# Autodesk Inventor assembly: BBM
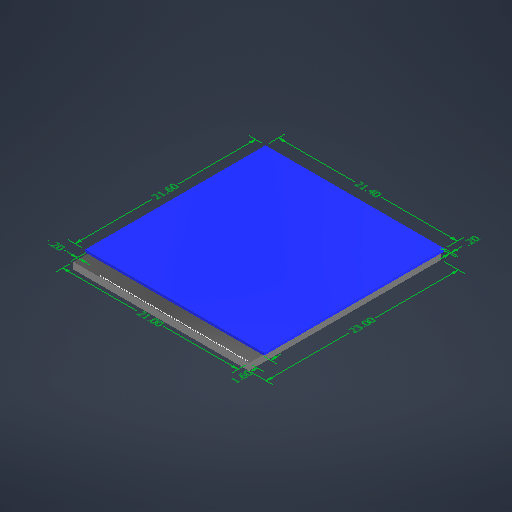
[picture p0: Inventor's stored thumbnail of the model, 512x512]
Saved by Autodesk Inventor 2027 (Build 310192060, 192F)
## iProperties
Created: 2022-02-01
Part Number: BBM
Document SubType Name: Assembly
Designer: Caleb
Author: Caleb
## Documents named in this file (4)
- C:\Users\cfang\Desktop\nebraska-silicon-lab\Hardware\ETL\modules\Tamale v1.7\BBM.iam
- C:\Users\cfang\Desktop\nebraska-silicon-lab\Hardware\ETL\modules\Tamale v1.7\ETL Sensor.ipt
- C:\Users\cfang\Desktop\nebraska-silicon-lab\Hardware\ETL\modules\Tamale v1.7\bump bond.ipt
- C:\Users\cfang\Desktop\nebraska-silicon-lab\Hardware\ETL\modules\Tamale v1.7\ETROC2.ipt
## Components (258 placed, 3 different names)
1. ETL Sensor:1 — Tangent:1, Tangent:2, Tangent:3, Flush:1, Flush:2, Mate:1
2. ETROC2:1 — Flush:1, Flush:2, Mate:1
3. bump bond:1 — Tangent:1, Tangent:2, Tangent:3
4. bump bond:2
5. bump bond:3
6. bump bond:4
7. bump bond:5
8. bump bond:6
9. bump bond:7
10. bump bond:8
11. bump bond:9
12. bump bond:10
13. bump bond:11
14. bump bond:12
15. bump bond:13
16. bump bond:14
17. bump bond:15
18. bump bond:16
19. bump bond:17
20. bump bond:18
21. bump bond:19
22. bump bond:20
23. bump bond:21
24. bump bond:22
25. bump bond:23
26. bump bond:24
27. bump bond:25
28. bump bond:26
29. bump bond:27
30. bump bond:28
31. bump bond:29
32. bump bond:30
33. bump bond:31
34. bump bond:32
35. bump bond:33
36. bump bond:34
37. bump bond:35
38. bump bond:36
39. bump bond:37
40. bump bond:38
41. bump bond:39
42. bump bond:40
43. bump bond:41
44. bump bond:42
45. bump bond:43
46. bump bond:44
47. bump bond:45
48. bump bond:46
49. bump bond:47
50. bump bond:48
51. bump bond:49
52. bump bond:50
53. bump bond:51
54. bump bond:52
55. bump bond:53
56. bump bond:54
57. bump bond:55
58. bump bond:56
59. bump bond:57
60. bump bond:58
61. bump bond:59
62. bump bond:60
63. bump bond:61
64. bump bond:62
65. bump bond:63
66. bump bond:64
67. bump bond:65
68. bump bond:66
69. bump bond:67
70. bump bond:68
71. bump bond:69
72. bump bond:70
73. bump bond:71
74. bump bond:72
75. bump bond:73
76. bump bond:74
77. bump bond:75
78. bump bond:76
79. bump bond:77
80. bump bond:78
81. bump bond:79
82. bump bond:80
83. bump bond:81
84. bump bond:82
85. bump bond:83
86. bump bond:84
87. bump bond:85
88. bump bond:86
89. bump bond:87
90. bump bond:88
91. bump bond:89
92. bump bond:90
93. bump bond:91
94. bump bond:92
95. bump bond:93
96. bump bond:94
97. bump bond:95
98. bump bond:96
99. bump bond:97
100. bump bond:98
101. bump bond:99
102. bump bond:100
103. bump bond:101
104. bump bond:102
105. bump bond:103
106. bump bond:104
107. bump bond:105
108. bump bond:106
109. bump bond:107
110. bump bond:108
111. bump bond:109
112. bump bond:110
113. bump bond:111
114. bump bond:112
115. bump bond:113
116. bump bond:114
117. bump bond:115
118. bump bond:116
119. bump bond:117
120. bump bond:118
121. bump bond:119
122. bump bond:120
123. bump bond:121
124. bump bond:122
125. bump bond:123
126. bump bond:124
127. bump bond:125
128. bump bond:126
129. bump bond:127
130. bump bond:128
131. bump bond:129
132. bump bond:130
133. bump bond:131
134. bump bond:132
135. bump bond:133
136. bump bond:134
137. bump bond:135
138. bump bond:136
139. bump bond:137
140. bump bond:138
141. bump bond:139
142. bump bond:140
143. bump bond:141
144. bump bond:142
145. bump bond:143
146. bump bond:144
147. bump bond:145
148. bump bond:146
149. bump bond:147
150. bump bond:148
151. bump bond:149
152. bump bond:150
153. bump bond:151
154. bump bond:152
155. bump bond:153
156. bump bond:154
157. bump bond:155
158. bump bond:156
159. bump bond:157
160. bump bond:158
161. bump bond:159
162. bump bond:160
163. bump bond:161
164. bump bond:162
165. bump bond:163
166. bump bond:164
167. bump bond:165
168. bump bond:166
169. bump bond:167
170. bump bond:168
171. bump bond:169
172. bump bond:170
173. bump bond:171
174. bump bond:172
175. bump bond:173
176. bump bond:174
177. bump bond:175
178. bump bond:176
179. bump bond:177
180. bump bond:178
181. bump bond:179
182. bump bond:180
183. bump bond:181
184. bump bond:182
185. bump bond:183
186. bump bond:184
187. bump bond:185
188. bump bond:186
189. bump bond:187
190. bump bond:188
191. bump bond:189
192. bump bond:190
193. bump bond:191
194. bump bond:192
195. bump bond:193
196. bump bond:194
197. bump bond:195
198. bump bond:196
199. bump bond:197
200. bump bond:198
201. bump bond:199
202. bump bond:200
203. bump bond:201
204. bump bond:202
205. bump bond:203
206. bump bond:204
207. bump bond:205
208. bump bond:206
209. bump bond:207
210. bump bond:208
211. bump bond:209
212. bump bond:210
213. bump bond:211
214. bump bond:212
215. bump bond:213
216. bump bond:214
217. bump bond:215
218. bump bond:216
219. bump bond:217
220. bump bond:218
221. bump bond:219
222. bump bond:220
223. bump bond:221
224. bump bond:222
225. bump bond:223
226. bump bond:224
227. bump bond:225
228. bump bond:226
229. bump bond:227
230. bump bond:228
231. bump bond:229
232. bump bond:230
233. bump bond:231
234. bump bond:232
235. bump bond:233
236. bump bond:234
237. bump bond:235
238. bump bond:236
239. bump bond:237
240. bump bond:238
241. bump bond:239
242. bump bond:240
243. bump bond:241
244. bump bond:242
245. bump bond:243
246. bump bond:244
247. bump bond:245
248. bump bond:246
249. bump bond:247
250. bump bond:248
251. bump bond:249
252. bump bond:250
253. bump bond:251
254. bump bond:252
255. bump bond:253
256. bump bond:254
257. bump bond:255
258. bump bond:256
## Component patterns: (256 elements, first: bump bond:1)
## Relationships (6: Tangent 3, Flush 2, Mate 1)
- Tangent:1: ETL Sensor:1 ↔ bump bond:1
- Tangent:2 (-0.65 mm): ETL Sensor:1 ↔ bump bond:1
- Tangent:3 (-0.65 mm): ETL Sensor:1 ↔ bump bond:1
- Flush:1 (0.2 mm): ETL Sensor:1 ↔ ETROC2:1
- Flush:2 (0.2 mm): ETL Sensor:1 ↔ ETROC2:1
- Mate:1 (0.08 mm): ETL Sensor:1 ↔ ETROC2:1
